# Autodesk Inventor assembly: MODI
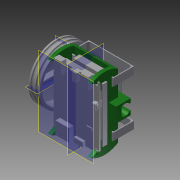
[picture p0: Inventor's stored thumbnail of the model, 180x180]
Saved by Autodesk Inventor 2013 (Build 170138000, 138)
## iProperties
Created: 2013-04-30
Part Number: MODI
Document SubType Name: Assembly
Designer: otrab
Author: otrab
## Documents named in this file (7)
- C:\Users\otrab\Documents\GitHub\modi\Hardware\inventor 2013\MODI.iam
- C:\Users\otrab\Documents\GitHub\modi\Hardware\inventor 2013\Chasis.ipt
- C:\Users\otrab\Documents\GitHub\modi\Hardware\inventor 2013\bateria.ipt
- C:\Users\otrab\Documents\GitHub\modi\Hardware\inventor 2013\fio.ipt
- C:\Users\otrab\Documents\GitHub\modi\Hardware\inventor 2013\lipoRiderPro.ipt
- C:\Users\otrab\Documents\GitHub\modi\Hardware\inventor 2013\Rueda.ipt
- C:\Users\otrab\Documents\GitHub\modi\Hardware\inventor 2013\tapa.ipt
## Components (7 placed, 6 different names)
1. Chasis:1 — Mate:3, Mate:4, Mate:5
2. bateria:1
3. fio:1 — Mate:3, Mate:4
4. lipoRiderPro:1 — Mate:5
5. Rueda:1
6. Rueda:2
7. tapa:1
## Relationships (3: Mate 3)
- Mate:3: Chasis:1 ↔ fio:1
- Mate:4: Chasis:1 ↔ fio:1
- Mate:5: Chasis:1 ↔ lipoRiderPro:1
